# Autodesk Inventor assembly: masbro
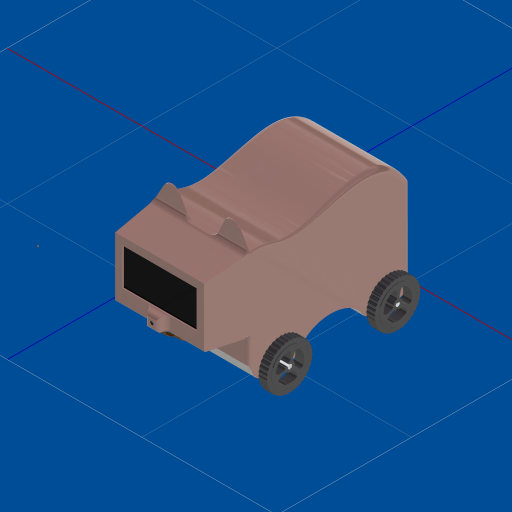
[picture p0: Inventor's stored thumbnail of the model, 512x512]
Saved by Autodesk Inventor 2023.1 (Build 271208000, 208)
## iProperties
Created: 2023-05-31
Part Number: masbro
Document SubType Name: Assembly
Designer: nara atthama
Author: nara atthama
## Documents named in this file (10)
- C:\Users\naraa\OneDrive - Universitas Airlangga\Dokumen\kuliah\MATKUL\sem6\TopSus\masbrobot\model\masbro.iam
- C:\Users\naraa\OneDrive - Universitas Airlangga\Dokumen\kuliah\MATKUL\sem6\TopSus\masbrobot\model\N20.iam
- C:\Users\naraa\OneDrive - Universitas Airlangga\Dokumen\kuliah\MATKUL\sem6\TopSus\masbrobot\model\top_case.ipt
- C:\Users\naraa\OneDrive - Universitas Airlangga\Dokumen\kuliah\MATKUL\sem6\TopSus\masbrobot\model\N20-Wheel\Llanta.ipt
- C:\Users\naraa\OneDrive - Universitas Airlangga\Dokumen\kuliah\MATKUL\sem6\TopSus\masbrobot\model\oled-2-42-v-4-1-1.snapshot.3\V2 Geometry.ipt
- C:\Users\naraa\OneDrive - Universitas Airlangga\Dokumen\kuliah\MATKUL\sem6\TopSus\masbrobot\model\rod.ipt
- C:\Users\naraa\OneDrive - Universitas Airlangga\Dokumen\kuliah\MATKUL\sem6\TopSus\masbrobot\model\lego-compatible-ov-camera-holder-with-long-cable-camera-1.snapshot.11\Long-cable-ov9655.iam
- C:\Users\naraa\OneDrive - Universitas Airlangga\Dokumen\kuliah\MATKUL\sem6\TopSus\masbrobot\model\cover.ipt
- C:\Users\naraa\OneDrive - Universitas Airlangga\Dokumen\kuliah\MATKUL\sem6\TopSus\masbrobot\model\cover_bottom.ipt
- C:\Users\naraa\OneDrive - Universitas Airlangga\Dokumen\kuliah\MATKUL\sem6\TopSus\masbrobot\model\electric_asm.iam
## Components (13 placed, 11 different names)
1. top_case:1 — Mate:6, Mate:7, Mate:8, Flush:3, Flush:4, Mate:12, Mate:13, Mate:14, Mate:15, Flush:8, Flush:9, Mate:16, Mate:17, Flush:10, Mate:18, Mate:19, Mate:20, Mate:21
2. V2 Geometry:1 — Mate:8, Flush:3, Flush:4
3. Llanta:3 — Flush:5, Mate:10
4. rod:1 — Flush:5, Mate:10, Mate:11, Flush:6, Mate:13
5. Llanta:4 — Mate:11, Flush:6, Flush:7
6. Long-cable-ov9655:1 [sub-assembly] — Mate:14, Mate:15
7. cover:1 — Flush:8, Flush:9, Mate:16
8. cover_bottom:1 — Mate:17, Flush:10, Mate:18
9. electric_asm:1 [sub-assembly] — Mate:19, Mate:20, Mate:21
10. N20:1 [sub-assembly] — Flush:1, Mate:3, Mate:7, Mate:12
11. N20:2 [sub-assembly] — Flush:2, Mate:5, Mate:6
12. wheel — Flush:2, Mate:5, Mate:9, Flush:7
13. wheel2 — Flush:1, Mate:3, Mate:9
## Relationships (28: Mate 18, Flush 10)
- Flush:1: N20:1 ↔ wheel2
- Mate:3: N20:1 ↔ wheel2
- Flush:2: N20:2 ↔ wheel
- Mate:5: N20:2 ↔ wheel
- Mate:6: top_case:1 ↔ N20:2
- Mate:7: top_case:1 ↔ N20:1
- Mate:8: top_case:1 ↔ V2 Geometry:1
- Flush:3: top_case:1 ↔ V2 Geometry:1
- Flush:4: top_case:1 ↔ V2 Geometry:1
- Mate:9: wheel ↔ wheel2
- Flush:5: Llanta:3 ↔ rod:1
- Mate:10: Llanta:3 ↔ rod:1
- Mate:11: rod:1 ↔ Llanta:4
- Flush:6: rod:1 ↔ Llanta:4
- Mate:12: top_case:1 ↔ N20:1
- Mate:13: top_case:1 ↔ rod:1
- Flush:7: Llanta:4 ↔ wheel
- Mate:14: top_case:1 ↔ Long-cable-ov9655:1
- Mate:15: top_case:1 ↔ Long-cable-ov9655:1
- Flush:8: top_case:1 ↔ cover:1
- Flush:9: top_case:1 ↔ cover:1
- Mate:16: top_case:1 ↔ cover:1
- Mate:17: top_case:1 ↔ cover_bottom:1
- Flush:10: top_case:1 ↔ cover_bottom:1
- Mate:18: top_case:1 ↔ cover_bottom:1
- Mate:19: top_case:1 ↔ electric_asm:1
- Mate:20 (1 mm): top_case:1 ↔ electric_asm:1
- Mate:21: top_case:1 ↔ electric_asm:1
